# Autodesk Inventor assembly: electronics_box
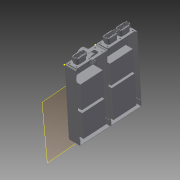
[picture p0: Inventor's stored thumbnail of the model, 180x180]
Saved by Autodesk Inventor 2015 (Build 190159000, 159)
## iProperties
Created: 2015-10-09
Part Number: electronics_box
Description: insert description/title
Document SubType Name: Assembly
Designer: c3132704
Part Category: insert part category and press enter to fill value
Author: c3132704
## Documents named in this file (7)
- C:\Users\c3132704\Documents\GitHub\CAD\electronics_box.iam
- C:\Users\c3132704\Documents\GitHub\CAD\stig.ipt
- C:\Users\c3132704\Documents\GitHub\CAD\fart.ipt
- C:\Users\c3132704\Documents\GitHub\CAD\solenoid_dvr.ipt
- C:\Users\c3132704\Documents\GitHub\CAD\halfbox.ipt
- C:\Users\c3132704\Documents\GitHub\CAD\Imported Components\c-dtm04-12pa-l012-99-3d\c-dtm04-12pa-l012-99-3d_2.ipt
- C:\Users\c3132704\Documents\GitHub\CAD\Imported Components\HDP_18_8\HDP_18_8.ipt
## Components (10 placed, 6 different names)
1. halfbox:1 — Flush:1, Mate:3, Mate:4, Mate:5, Mate:6, Flush:2, Mate:7, Flush:3, Mate:8, Angle:1, Angle:2, Angle:3, Angle:4, Flush:4, Flush:5, Mate:9, Mate:10, Mate:11
2. halfbox:2 — Flush:2, Mate:7, Flush:3, Mate:13
3. stig:1 — Mate:5, Angle:4
4. fart:1 — Mate:8, Angle:3
5. solenoid_dvr:1 — Mate:3, Angle:1
6. solenoid_dvr:2 — Mate:4, Mate:6, Angle:2
7. c-dtm04-12pa-l012-99-3d_2:1 — Flush:5, Mate:11
8. c-dtm04-12pa-l012-99-3d_2:2 — Flush:4, Mate:10, Mate:12
9. c-dtm04-12pa-l012-99-3d_2:3 — Flush:1, Mate:9, Mate:12
10. HDP_18_8:1 — Mate:13
## Relationships (20: Mate 11, Flush 5, Angle 4)
- Flush:1: halfbox:1 ↔ c-dtm04-12pa-l012-99-3d_2:3
- Mate:3: halfbox:1 ↔ solenoid_dvr:1
- Mate:4: halfbox:1 ↔ solenoid_dvr:2
- Mate:5: halfbox:1 ↔ stig:1
- Mate:6: halfbox:1 ↔ solenoid_dvr:2
- Flush:2: halfbox:1 ↔ halfbox:2
- Mate:7: halfbox:1 ↔ halfbox:2
- Flush:3: halfbox:1 ↔ halfbox:2
- Mate:8: halfbox:1 ↔ fart:1
- Angle:1 (0 deg): halfbox:1 ↔ solenoid_dvr:1
- Angle:2 (0 deg): halfbox:1 ↔ solenoid_dvr:2
- Angle:3 (0 deg): halfbox:1 ↔ fart:1
- Angle:4 (0 deg): halfbox:1 ↔ stig:1
- Flush:4: halfbox:1 ↔ c-dtm04-12pa-l012-99-3d_2:2
- Flush:5: halfbox:1 ↔ c-dtm04-12pa-l012-99-3d_2:1
- Mate:9: halfbox:1 ↔ c-dtm04-12pa-l012-99-3d_2:3
- Mate:10: halfbox:1 ↔ c-dtm04-12pa-l012-99-3d_2:2
- Mate:11: halfbox:1 ↔ c-dtm04-12pa-l012-99-3d_2:1
- Mate:12: c-dtm04-12pa-l012-99-3d_2:2 ↔ c-dtm04-12pa-l012-99-3d_2:3
- Mate:13: halfbox:2 ↔ HDP_18_8:1
